# Autodesk Inventor assembly: colsonwgeelwithhub
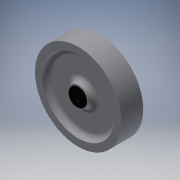
[picture p0: Inventor's stored thumbnail of the model, 180x180]
Saved by Autodesk Inventor 2018 (Build 220112000, 112)
## iProperties
Created: 2018-07-02
Part Number: colsonwgeelwithhub
Document SubType Name: Assembly
Designer: s-2512711
Author: s-2512711
## Documents named in this file (3)
- C:\Users\s-2512711\Desktop\New folder\colsonwgeelwithhub.iam
- C:\Users\s-2512711\Desktop\New folder\Colson_Live_Hub_217-3430.ipt
- C:\Users\s-2512711\Desktop\New folder\Part7.ipt
## Components (2 placed, 2 different names)
1. Colson_Live_Hub_217-3430:1 — Mate:1, Mate:2, Rotation:1
2. Part7:1 — Mate:1, Mate:2, Rotation:1
## Relationships (3: Mate 2, RelateRotation 1)
- Mate:1: Colson_Live_Hub_217-3430:1 ↔ Part7:1
- Mate:2: Colson_Live_Hub_217-3430:1 ↔ Part7:1
- Rotation:1 [RelateRotation] (1 ul): Colson_Live_Hub_217-3430:1 ↔ Part7:1
